# Autodesk Inventor assembly: Support_Link_COG
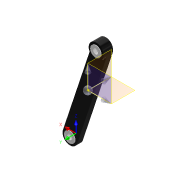
[picture p0: Inventor's stored thumbnail of the model, 180x180]
Saved by Autodesk Inventor 2022 (Build 260153000, 153)
## iProperties
Created: 2022-10-18
Part Number: Support_Link_COG
Document SubType Name: Assembly
Designer: alexw
Mass: 71.2897 g
Surface Area: 198.559 cm^2
Volume: 46.9153 cm^3
Author: alexw
## Documents named in this file (3)
- C:\Users\alexw\Documents\Inventor\Projects\03_CurrentProjects\MasterThesis\PSM_V1_Rillenkugellager\COG\Support_Link_COG.iam
- C:\Users\alexw\Documents\Inventor\Projects\03_CurrentProjects\MasterThesis\PSM_V1_Rillenkugellager\ParallelMechanismus_Support_Rillenkugellager.iam
- C:\Users\alexw\Documents\Inventor\Projects\03_CurrentProjects\MasterThesis\PSM_V1_Rillenkugellager\SpringCompensation_Innside_SupportPart.ipt
## Components (2 placed, 2 different names)
1. ParallelMechanismus_Support_Rillenkugellager:1 [sub-assembly] — Passend:3, Passend:4, Winkel:1
2. SpringCompensation_Innside_SupportPart:1
## Relationships (5: Mate 4, Angle 1)
- [Mate]: ParallelMechanismus_Support_Rillenkugellager:1 ↔ SpringCompensation_Innside_SupportPart:1
- [Mate]: ParallelMechanismus_Support_Rillenkugellager:1 ↔ SpringCompensation_Innside_SupportPart:1
- Passend:3 [Mate]: ParallelMechanismus_Support_Rillenkugellager:1
- Passend:4 [Mate]: ParallelMechanismus_Support_Rillenkugellager:1
- Winkel:1 [Angle] (251.8 deg): ParallelMechanismus_Support_Rillenkugellager:1
